# Autodesk Inventor assembly: FrisbeeShooter
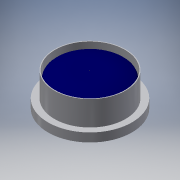
[picture p0: Inventor's stored thumbnail of the model, 180x180]
Saved by Autodesk Inventor 2016 (Build 200138000, 138)
## iProperties
Created: 2015-07-20
Part Number: FrisbeeShooter
Document SubType Name: Assembly
Designer: steele
Mass: 805.932 g
Surface Area: 5289.21 cm^2
Volume: 1648.45 cm^3
Density: 0.488903 g/cm^3
Author: steele
## Documents named in this file (4)
- C:\snobotics\CAD-Development\robSteele\FRC 2013 Ultimate Ascent\FrisbeeShooter.iam
- C:\snobotics\CAD-Development\robSteele\FRC 2013 Ultimate Ascent\FrisbeeHopper.ipt
- C:\snobotics\ptc\FRC 2013 Ultimate Acsent\FRC_KOP\2013_frc_kop\Black Tote\53214-b_2013.ipt
- C:\snobotics\CAD-Development\robSteele\FRC 2013 Ultimate Ascent\DiskCam.ipt
## Components (3 placed, 3 different names)
1. FrisbeeHopper:1 — Insert:1, Insert:2
2. 53214-b_2013:1 — Insert:1
3. DiskCam:1 — Insert:2
## Relationships (2: Insert 2)
- Insert:1: FrisbeeHopper:1 ↔ 53214-b_2013:1
- Insert:2 (-6.35 mm): FrisbeeHopper:1 ↔ DiskCam:1
